# Autodesk Inventor assembly: eLECTRONICS-ENCLOSURE
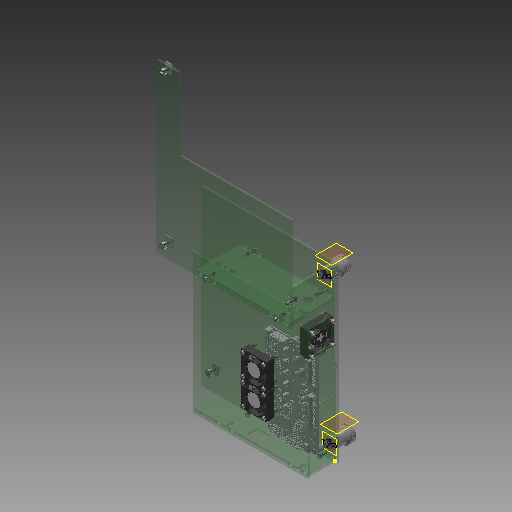
[picture p0: Inventor's stored thumbnail of the model, 512x512]
Saved by Autodesk Inventor 2017 (Build 210142000, 142)
## iProperties
Created: 2016-07-27
Part Number: eLECTRONICS-ENCLOSURE
Document SubType Name: Assembly
Designer: User
Author: User
## Documents named in this file (19)
- C:\All INVENTOR\SL-Inventor\SL-Beast 3D Printer\eLECTRONICS-ENCLOSURE.iam
- C:\All INVENTOR\SL-Inventor\SL-Beast 3D Printer\EE PSU TOP.ipt
- C:\All INVENTOR\SL-Inventor\SL-Beast 3D Printer\EE Top.ipt
- C:\All INVENTOR\SL-Inventor\SL-Beast 3D Printer\EE Side.ipt
- C:\All INVENTOR\SL-Inventor\SL-Beast 3D Printer\EE Side 2.ipt
- C:\All INVENTOR\SL-Inventor\SL-Beast 3D Printer\EE Base.ipt
- C:\All INVENTOR\SL-Inventor\SL-Beast 3D Printer\EE-Rear.ipt
- C:\All INVENTOR\SL-Inventor\SL-Beast 3D Printer\EE Foot.ipt
- C:\All INVENTOR\SL-Inventor\SL-Beast 3D Printer\en-US\ANSI B18.3.1M(6)\ANSI B18.3.1M - M3x0.5 x 16(1).ipt
- C:\All INVENTOR\SL-Inventor\SL-Beast 3D Printer\en-US\ANSI B18.3.1M(6)\ANSI B18.3.1M - M3x0.5 x 12(1).ipt
- C:\All INVENTOR\SL-Inventor\SL-Beast 3D Printer\en-US\CSN EN 24 036\CSN EN 24 036 - M3.ipt
- C:\All INVENTOR\SL-Inventor\SL-Beast 3D Printer\en-US\ANSI B18.3.1M(6)\ANSI B18.3.1M - M5x0.8 x 12(1).ipt
- C:\All INVENTOR\SL-Inventor\SL-Beast 3D Printer\40mm_fan_MIR.ipt
- C:\All INVENTOR\SL-Inventor\SL-Beast 3D Printer\en-US\ANSI B18.3.1M(6)\ANSI B18.3.1M - M3x0.5 x 20(1).ipt
- C:\All INVENTOR\SL-Inventor\SL-Beast 3D Printer\en-US\JIS B 1251 C1 (1L 1H)\JIS B 1251  - 3 1L.ipt
- C:\All INVENTOR\SL-Inventor\SL-Beast 3D Printer\8mm Rumba Spacer.ipt
- C:\All INVENTOR\SL-Inventor\SL-Beast 3D Printer\RUMBA+PCB.ipt
- C:\All INVENTOR\SL-Inventor\SL-Beast 3D Printer\Fanwithscrews.iam
- C:\All INVENTOR\SL-Inventor\SL-Beast 3D Printer\M5 Tee Nut-Generic_MIR_CPY_CPY.ipt
## Components (63 placed, 18 different names)
1. EE PSU TOP:1 — Mate:10, Mate:11, Mate:12, Mate:31, Mate:32, Mate:33, Mate:34, Mate:37, Mate:38, Insert:12, Insert:13, Mate:99
2. EE Top:1 — Mate:74, Mate:75, Mate:76, Mate:95, Mate:96
3. EE Front — Mate:1, Mate:2, Mate:3, Flush:1, Mate:20, Mate:22
4. EE Side 2:1 — Mate:4, Mate:5, Flush:1, Mate:24, Mate:26, Mate:40, Mate:45, Mate:46, Angle:1, Insert:14, Mate:74
5. EE Base:1 — Mate:1, Mate:2, Mate:3, Mate:4, Mate:5, Mate:6, Mate:8, Mate:9, Mate:13, Mate:14, Mate:15, Mate:16, Insert:2, Insert:6, Insert:7, Insert:8, Insert:10, Insert:11, Mate:59, Insert:15, Insert:16, Mate:61, Flush:5, Mate:64, Mate:65, Mate:66, Angle:2, Mate:101, Mate:102, Mate:103
6. EE-Rear:1 — Mate:6, Mate:8, Mate:9, Mate:10, Mate:11, Mate:12, Mate:28, Mate:30, Mate:42, Mate:44, Mate:75, Mate:76
7. EE Foot:1 — Mate:13, Mate:16, Mate:104, Insert:17
8. EE Foot:2 — Mate:14, Mate:15, Mate:17, Mate:18
9. RUMBA+PCB:2
10. Forged Socket Head Cap Screw - Metric M3x0.5 x 20:1 — Mate:17, Mate:18, Mate:58, Mate:60
11. Forged Socket Head Cap Screw - Metric M3x0.5 x 12:1 — Insert:2, Mate:19
12. Forged Socket Head Cap Screw - Metric M3x0.5 x 12:5 — Insert:6, Mate:27
13. Forged Socket Head Cap Screw - Metric M3x0.5 x 12:6 — Insert:7, Mate:25
14. Forged Socket Head Cap Screw - Metric M3x0.5 x 12:7 — Insert:8, Mate:29
15. Forged Socket Head Cap Screw - Metric M3x0.5 x 12:9 — Insert:10, Mate:23
16. Forged Socket Head Cap Screw - Metric M3x0.5 x 12:10 — Insert:11, Mate:21
17. CSN EN 24036 M3:1 — Mate:19, Mate:20
18. CSN EN 24036 M3:2 — Mate:21, Mate:22
19. CSN EN 24036 M3:3 — Mate:23, Mate:24
20. CSN EN 24036 M3:4 — Mate:25, Mate:26
21. CSN EN 24036 M3:5 — Mate:27, Mate:28
22. CSN EN 24036 M3:6 — Mate:29, Mate:30
23. Forged Socket Head Cap Screw - Metric M3x0.5 x 12:11 — Mate:31, Mate:32, Mate:39
24. Forged Socket Head Cap Screw - Metric M3x0.5 x 12:12 — Mate:33, Mate:34, Mate:41
25. Forged Socket Head Cap Screw - Metric M3x0.5 x 12:14 — Mate:37, Mate:38, Mate:43
26. CSN EN 24036 M3:15
27. CSN EN 24036 M3:16
28. CSN EN 24036 M3:17
29. CSN EN 24036 M3:18
30. Forged Socket Head Cap Screw - Metric M5x0.8 x 12:1 — Insert:12, Mate:98
31. Forged Socket Head Cap Screw - Metric M5x0.8 x 12:2 — Insert:13, Mate:97
32. CSN EN 24036 M3:7 — Mate:39, Mate:40
33. CSN EN 24036 M3:8 — Mate:41, Mate:42
34. CSN EN 24036 M3:9 — Mate:43, Mate:44
35. 40mm_fan_MIR:1 — Mate:45, Mate:46, Angle:1, Mate:47, Mate:48, Mate:49, Mate:51, Mate:53, Mate:55, Mate:57
36. Forged Socket Head Cap Screw - Metric M3x0.5 x 16:2 — Insert:14, Flush:2, Flush:4, Mate:52
37. Forged Socket Head Cap Screw - Metric M3x0.5 x 16:3 — Mate:49, Flush:3, Mate:56
38. Forged Socket Head Cap Screw - Metric M3x0.5 x 16:4 — Mate:47, Flush:3, Flush:4, Mate:54
39. Forged Socket Head Cap Screw - Metric M3x0.5 x 16:5 — Mate:48, Flush:2, Mate:50
40. CSN EN 24036 M3:10 — Mate:50, Mate:51
41. CSN EN 24036 M3:11 — Mate:52, Mate:53
42. CSN EN 24036 M3:12 — Mate:54, Mate:55
43. CSN EN 24036 M3:13 — Mate:56, Mate:57
44. JIS B 1251 Class 1 (1L/1H) 3 1L:1 — Mate:58, Mate:59
45. JIS B 1251 Class 1 (1L/1H) 3 1L:3 — Insert:15
46. JIS B 1251 Class 1 (1L/1H) 3 1L:2 — Insert:16
47. CSN EN 24036 M3:14 — Mate:60, Mate:61
48. 8mm Rumba Spacer:1 — Flush:5, Flush:7, Flush:8, Mate:70
49. 8mm Rumba Spacer:2 — Mate:64, Flush:6, Flush:7, Mate:72
50. 8mm Rumba Spacer:4 — Mate:65, Flush:6, Mate:73
51. 8mm Rumba Spacer:5 — Flush:8, Mate:66, Mate:67, Mate:68
52. RUMBA+PCB:1 — Mate:67, Angle:2, Mate:69, Mate:71
53. Forged Socket Head Cap Screw - Metric M3x0.5 x 16:6 — Flush:10, Mate:70
54. Forged Socket Head Cap Screw - Metric M3x0.5 x 16:7 — Mate:68, Mate:69
55. Forged Socket Head Cap Screw - Metric M3x0.5 x 16:8 — Flush:9, Flush:10, Mate:71, Mate:72
56. Forged Socket Head Cap Screw - Metric M3x0.5 x 16:9 — Flush:9, Mate:73
57. Fanwithscrews:1 [sub-assembly] — Flush:11
58. Fanwithscrews:2 [sub-assembly] — Mate:95, Flush:11, Mate:96
59. M5 Tee Nut-Generic_MIR_CPY_CPY:1 — Mate:97, Flush:12
60. M5 Tee Nut-Generic_MIR_CPY_CPY:2 — Mate:98, Flush:12, Mate:99
61. Forged Socket Head Cap Screw - Metric M5x0.8 x 12:3 — Mate:101, Mate:102
62. M5 Tee Nut-Generic_MIR_CPY_CPY:3 — Mate:103
63. Forged Socket Head Cap Screw - Metric M3x0.5 x 20:2 — Mate:104, Insert:17
## Relationships (125: Mate 99, Flush 12, Insert 12, Angle 2)
- Mate:1: EE Front ↔ EE Base:1
- Mate:2: EE Front ↔ EE Base:1
- Mate:3: EE Front ↔ EE Base:1
- Mate:4: EE Side 2:1 ↔ EE Base:1
- Mate:5: EE Side 2:1 ↔ EE Base:1
- Flush:1: EE Front ↔ EE Side 2:1
- Mate:6: EE Base:1 ↔ EE-Rear:1
- Mate:8: EE Base:1 ↔ EE-Rear:1
- Mate:9: EE Base:1 ↔ EE-Rear:1
- Mate:10: EE PSU TOP:1 ↔ EE-Rear:1
- Mate:11: EE PSU TOP:1 ↔ EE-Rear:1
- Mate:12: EE PSU TOP:1 ↔ EE-Rear:1
- Mate:13: EE Base:1 ↔ EE Foot:1
- Mate:14: EE Base:1 ↔ EE Foot:2
- Mate:15: EE Base:1 ↔ EE Foot:2
- Mate:16: EE Base:1 ↔ EE Foot:1
- Mate:17: EE Foot:2 ↔ Forged Socket Head Cap Screw - Metric M3x0.5 x 20:1
- Mate:18: EE Foot:2 ↔ Forged Socket Head Cap Screw - Metric M3x0.5 x 20:1
- Insert:2: EE Base:1 ↔ Forged Socket Head Cap Screw - Metric M3x0.5 x 12:1
- Insert:6: EE Base:1 ↔ Forged Socket Head Cap Screw - Metric M3x0.5 x 12:5
- Insert:7: EE Base:1 ↔ Forged Socket Head Cap Screw - Metric M3x0.5 x 12:6
- Insert:8: EE Base:1 ↔ Forged Socket Head Cap Screw - Metric M3x0.5 x 12:7
- Insert:10: EE Base:1 ↔ Forged Socket Head Cap Screw - Metric M3x0.5 x 12:9
- Insert:11: EE Base:1 ↔ Forged Socket Head Cap Screw - Metric M3x0.5 x 12:10
- Mate:19: Forged Socket Head Cap Screw - Metric M3x0.5 x 12:1 ↔ CSN EN 24036 M3:1
- Mate:20: EE Front ↔ CSN EN 24036 M3:1
- Mate:21: Forged Socket Head Cap Screw - Metric M3x0.5 x 12:10 ↔ CSN EN 24036 M3:2
- Mate:22: EE Front ↔ CSN EN 24036 M3:2
- Mate:23: Forged Socket Head Cap Screw - Metric M3x0.5 x 12:9 ↔ CSN EN 24036 M3:3
- Mate:24: EE Side 2:1 ↔ CSN EN 24036 M3:3
- Mate:25: Forged Socket Head Cap Screw - Metric M3x0.5 x 12:6 ↔ CSN EN 24036 M3:4
- Mate:26: EE Side 2:1 ↔ CSN EN 24036 M3:4
- Mate:27: Forged Socket Head Cap Screw - Metric M3x0.5 x 12:5 ↔ CSN EN 24036 M3:5
- Mate:28: EE-Rear:1 ↔ CSN EN 24036 M3:5
- Mate:29: Forged Socket Head Cap Screw - Metric M3x0.5 x 12:7 ↔ CSN EN 24036 M3:6
- Mate:30: EE-Rear:1 ↔ CSN EN 24036 M3:6
- Mate:31: EE PSU TOP:1 ↔ Forged Socket Head Cap Screw - Metric M3x0.5 x 12:11
- Mate:32: EE PSU TOP:1 ↔ Forged Socket Head Cap Screw - Metric M3x0.5 x 12:11
- Mate:33: EE PSU TOP:1 ↔ Forged Socket Head Cap Screw - Metric M3x0.5 x 12:12
- Mate:34: EE PSU TOP:1 ↔ Forged Socket Head Cap Screw - Metric M3x0.5 x 12:12
- Mate:37: EE PSU TOP:1 ↔ Forged Socket Head Cap Screw - Metric M3x0.5 x 12:14
- Mate:38: EE PSU TOP:1 ↔ Forged Socket Head Cap Screw - Metric M3x0.5 x 12:14
- Insert:12: EE PSU TOP:1 ↔ Forged Socket Head Cap Screw - Metric M5x0.8 x 12:1
- Insert:13: EE PSU TOP:1 ↔ Forged Socket Head Cap Screw - Metric M5x0.8 x 12:2
- Mate:39: Forged Socket Head Cap Screw - Metric M3x0.5 x 12:11 ↔ CSN EN 24036 M3:7
- Mate:40: EE Side 2:1 ↔ CSN EN 24036 M3:7
- Mate:41: Forged Socket Head Cap Screw - Metric M3x0.5 x 12:12 ↔ CSN EN 24036 M3:8
- Mate:42: EE-Rear:1 ↔ CSN EN 24036 M3:8
- Mate:43: Forged Socket Head Cap Screw - Metric M3x0.5 x 12:14 ↔ CSN EN 24036 M3:9
- Mate:44: EE-Rear:1 ↔ CSN EN 24036 M3:9
- Mate:45: EE Side 2:1 ↔ 40mm_fan_MIR:1
- Mate:46: EE Side 2:1 ↔ 40mm_fan_MIR:1
- Angle:1 (0 deg): EE Side 2:1 ↔ 40mm_fan_MIR:1
- Insert:14: EE Side 2:1 ↔ Forged Socket Head Cap Screw - Metric M3x0.5 x 16:2
- Mate:47: 40mm_fan_MIR:1 ↔ Forged Socket Head Cap Screw - Metric M3x0.5 x 16:4
- Mate:48: 40mm_fan_MIR:1 ↔ Forged Socket Head Cap Screw - Metric M3x0.5 x 16:5
- Mate:49: 40mm_fan_MIR:1 ↔ Forged Socket Head Cap Screw - Metric M3x0.5 x 16:3
- Flush:2: Forged Socket Head Cap Screw - Metric M3x0.5 x 16:2 ↔ Forged Socket Head Cap Screw - Metric M3x0.5 x 16:5
- Flush:3: Forged Socket Head Cap Screw - Metric M3x0.5 x 16:3 ↔ Forged Socket Head Cap Screw - Metric M3x0.5 x 16:4
- Flush:4: Forged Socket Head Cap Screw - Metric M3x0.5 x 16:2 ↔ Forged Socket Head Cap Screw - Metric M3x0.5 x 16:4
- Mate:50: Forged Socket Head Cap Screw - Metric M3x0.5 x 16:5 ↔ CSN EN 24036 M3:10
- Mate:51: 40mm_fan_MIR:1 ↔ CSN EN 24036 M3:10
- Mate:52: Forged Socket Head Cap Screw - Metric M3x0.5 x 16:2 ↔ CSN EN 24036 M3:11
- Mate:53: 40mm_fan_MIR:1 ↔ CSN EN 24036 M3:11
- Mate:54: Forged Socket Head Cap Screw - Metric M3x0.5 x 16:4 ↔ CSN EN 24036 M3:12
- Mate:55: 40mm_fan_MIR:1 ↔ CSN EN 24036 M3:12
- Mate:56: Forged Socket Head Cap Screw - Metric M3x0.5 x 16:3 ↔ CSN EN 24036 M3:13
- Mate:57: 40mm_fan_MIR:1 ↔ CSN EN 24036 M3:13
- Mate:58: Forged Socket Head Cap Screw - Metric M3x0.5 x 20:1 ↔ JIS B 1251 Class 1 (1L/1H) 3 1L:1
- Mate:59: EE Base:1 ↔ JIS B 1251 Class 1 (1L/1H) 3 1L:1
- Insert:15: EE Base:1 ↔ JIS B 1251 Class 1 (1L/1H) 3 1L:3
- Insert:16: EE Base:1 ↔ JIS B 1251 Class 1 (1L/1H) 3 1L:2
- Mate:60: Forged Socket Head Cap Screw - Metric M3x0.5 x 20:1 ↔ CSN EN 24036 M3:14
- Mate:61: EE Base:1 ↔ CSN EN 24036 M3:14
- Flush:5: EE Base:1 ↔ 8mm Rumba Spacer:1
- Mate:64: EE Base:1 ↔ 8mm Rumba Spacer:2
- Mate:65: EE Base:1 ↔ 8mm Rumba Spacer:4
- Flush:6: 8mm Rumba Spacer:2 ↔ 8mm Rumba Spacer:4
- Flush:7: 8mm Rumba Spacer:1 ↔ 8mm Rumba Spacer:2
- Flush:8: 8mm Rumba Spacer:1 ↔ 8mm Rumba Spacer:5
- Mate:66: EE Base:1 ↔ 8mm Rumba Spacer:5
- Mate:67: 8mm Rumba Spacer:5 ↔ RUMBA+PCB:1
- Angle:2 (0 deg): EE Base:1 ↔ RUMBA+PCB:1
- Mate:68: 8mm Rumba Spacer:5 ↔ Forged Socket Head Cap Screw - Metric M3x0.5 x 16:7
- Mate:69: RUMBA+PCB:1 ↔ Forged Socket Head Cap Screw - Metric M3x0.5 x 16:7
- Flush:9: Forged Socket Head Cap Screw - Metric M3x0.5 x 16:8 ↔ Forged Socket Head Cap Screw - Metric M3x0.5 x 16:9
- Flush:10: Forged Socket Head Cap Screw - Metric M3x0.5 x 16:6 ↔ Forged Socket Head Cap Screw - Metric M3x0.5 x 16:8
- Mate:70: 8mm Rumba Spacer:1 ↔ Forged Socket Head Cap Screw - Metric M3x0.5 x 16:6
- Mate:71: RUMBA+PCB:1 ↔ Forged Socket Head Cap Screw - Metric M3x0.5 x 16:8
- Mate:72: 8mm Rumba Spacer:2 ↔ Forged Socket Head Cap Screw - Metric M3x0.5 x 16:8
- Mate:73: 8mm Rumba Spacer:4 ↔ Forged Socket Head Cap Screw - Metric M3x0.5 x 16:9
- Mate:74: EE Top:1 ↔ EE Side 2:1
- Mate:75: EE Top:1 ↔ EE-Rear:1
- Mate:76: EE Top:1 ↔ EE-Rear:1
- [Mate]: EE Top:1 ↔ Fanwithscrews:1
- [Mate]: EE Top:1 ↔ Fanwithscrews:1
- [Mate]: EE Top:1 ↔ Fanwithscrews:1
- [Mate]: EE Top:1 ↔ Fanwithscrews:1
- [Mate]: EE Top:1 ↔ Fanwithscrews:1
- [Mate]: EE Top:1 ↔ Fanwithscrews:1
- [Mate]: EE Top:1 ↔ Fanwithscrews:1
- [Mate]: EE Top:1 ↔ Fanwithscrews:1
- [Mate]: EE Top:1 ↔ Fanwithscrews:1
- [Mate]: EE Top:1 ↔ Fanwithscrews:1
- Mate:95: EE Top:1 ↔ Fanwithscrews:2
- Flush:11: Fanwithscrews:1 ↔ Fanwithscrews:2
- Mate:96: EE Top:1 ↔ Fanwithscrews:2
- Mate:97: Forged Socket Head Cap Screw - Metric M5x0.8 x 12:2 ↔ M5 Tee Nut-Generic_MIR_CPY_CPY:1
- Mate:98: Forged Socket Head Cap Screw - Metric M5x0.8 x 12:1 ↔ M5 Tee Nut-Generic_MIR_CPY_CPY:2
- Flush:12: M5 Tee Nut-Generic_MIR_CPY_CPY:1 ↔ M5 Tee Nut-Generic_MIR_CPY_CPY:2
- Mate:99 (3 mm): EE PSU TOP:1 ↔ M5 Tee Nut-Generic_MIR_CPY_CPY:2
- [Mate]: Forged Socket Head Cap Screw - Metric M5x0.8 x 12:3 ↔ M5 Tee Nut-Generic_MIR_CPY_CPY:3
- Mate:101: EE Base:1 ↔ Forged Socket Head Cap Screw - Metric M5x0.8 x 12:3
- Mate:102: EE Base:1 ↔ Forged Socket Head Cap Screw - Metric M5x0.8 x 12:3
- Mate:103 (3 mm): EE Base:1 ↔ M5 Tee Nut-Generic_MIR_CPY_CPY:3
- Mate:104: EE Foot:1 ↔ Forged Socket Head Cap Screw - Metric M3x0.5 x 20:2
- Insert:17: EE Foot:1 ↔ Forged Socket Head Cap Screw - Metric M3x0.5 x 20:2
- [Mate]: CSN EN 24036 M3:15 ↔ Forged Socket Head Cap Screw - Metric M3x0.5 x 16:8
- [Mate]: EE Base:1 ↔ CSN EN 24036 M3:15
- [Mate]: CSN EN 24036 M3:16 ↔ Forged Socket Head Cap Screw - Metric M3x0.5 x 16:9
- [Mate]: EE Base:1 ↔ CSN EN 24036 M3:16
- [Mate]: CSN EN 24036 M3:17 ↔ Forged Socket Head Cap Screw - Metric M3x0.5 x 16:7
- [Mate]: EE Base:1 ↔ CSN EN 24036 M3:17
- [Mate]: CSN EN 24036 M3:18 ↔ Forged Socket Head Cap Screw - Metric M3x0.5 x 16:6
- [Mate]: EE Base:1 ↔ CSN EN 24036 M3:18
## Named parameters: d238_d235 = 0 mm
